# Autodesk Inventor assembly: Connection rod
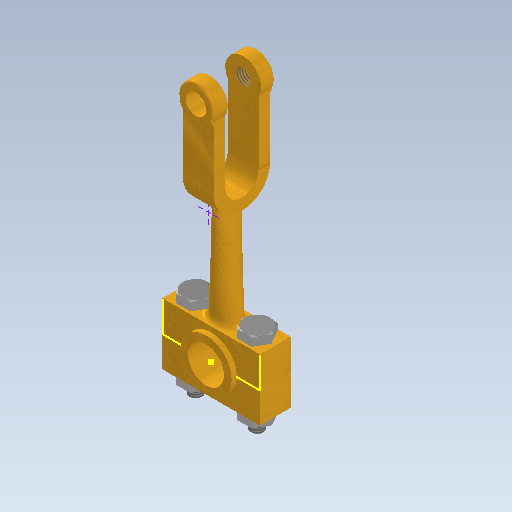
[picture p0: Inventor's stored thumbnail of the model, 512x512]
Saved by Autodesk Inventor 2020 (Build 240168000, 168)
## iProperties
Created: 2021-10-29
Part Number: Connection rod
Document SubType Name: Assembly
Designer: simon.erikssonwestl
Author: simon.erikssonwestl
## Documents named in this file (5)
- C:\Users\simon.erikssonwestl\Documents\Inventor\Ång\Assemblies\Connection rod.iam
- C:\Users\simon.erikssonwestl\Documents\Inventor\Ång\Part21.ipt
- C:\Users\simon.erikssonwestl\Documents\Inventor\Ång\Part22.ipt
- C:\Users\simon.erikssonwestl\Documents\Inventor\Content Center Files\R2020\en-US\AS 1474(1)\AS 1474 - M2,5(1).ipt
- C:\Users\simon.erikssonwestl\Documents\Inventor\Content Center Files\R2020\en-US\AS 1110\AS 1110 - M2,5 x 16.ipt
## Components (6 placed, 4 different names)
1. Part21:1 — Mate:1, Mate:2, Mate:3, Mate:4, Mate:5, Mate:6, Mate:7
2. Part22:1 — Mate:1, Mate:2, Mate:3, Mate:10, Mate:11
3. AS 1474 - Metric M2,5:1 — Mate:8, Mate:11
4. AS 1474 - Metric M2,5:2 — Mate:9, Mate:10
5. AS 1110 - Metric M2,5 x 16:1 — Mate:6, Mate:7, Mate:8
6. AS 1110 - Metric M2,5 x 16:2 — Mate:4, Mate:5, Mate:9
## Relationships (11: Mate 11)
- Mate:1: Part21:1 ↔ Part22:1
- Mate:2: Part21:1 ↔ Part22:1
- Mate:3: Part21:1 ↔ Part22:1
- Mate:4: Part21:1 ↔ AS 1110 - Metric M2,5 x 16:2
- Mate:5: Part21:1 ↔ AS 1110 - Metric M2,5 x 16:2
- Mate:6: Part21:1 ↔ AS 1110 - Metric M2,5 x 16:1
- Mate:7: Part21:1 ↔ AS 1110 - Metric M2,5 x 16:1
- Mate:8: AS 1474 - Metric M2,5:1 ↔ AS 1110 - Metric M2,5 x 16:1
- Mate:9: AS 1474 - Metric M2,5:2 ↔ AS 1110 - Metric M2,5 x 16:2
- Mate:10: Part22:1 ↔ AS 1474 - Metric M2,5:2
- Mate:11: Part22:1 ↔ AS 1474 - Metric M2,5:1
